# Autodesk Inventor assembly: montagem rolamento
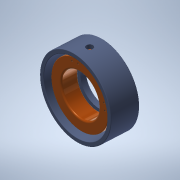
[picture p0: Inventor's stored thumbnail of the model, 180x180]
Saved by Autodesk Inventor 2020.4 (Build 244396000, 396)
## iProperties
Created: 2016-03-04
Part Number: montagem rolamento
Document SubType Name: Assembly
Designer: Everton
Author: Everton
## Documents named in this file (3)
- C:\Users\Alison\Documents\TCC\Desenhos e Montagem\desenhos e montagems inventor 15\MONTAGEM_ROLAMENTO.iam
- C:\Users\Alison\Documents\TCC\Desenhos e Montagem\desenhos e montagems inventor 15\ROLAMENTO_INFERIOR_BASE.ipt
- C:\Users\Alison\Documents\TCC\Desenhos e Montagem\desenhos e montagems inventor 15\ROLAMENTO_INFERIOR_INTERNO.ipt
## Components (2 placed, 2 different names)
1. ROLAMENTO_INFERIOR_BASE:1 — Mate:1, Mate:2
2. ROLAMENTO_INFERIOR_INTERNO:1 — Mate:1, Mate:2
## Relationships (2: Mate 2)
- Mate:1 (6 mm): ROLAMENTO_INFERIOR_BASE:1 ↔ ROLAMENTO_INFERIOR_INTERNO:1
- Mate:2: ROLAMENTO_INFERIOR_BASE:1 ↔ ROLAMENTO_INFERIOR_INTERNO:1
